# Autodesk Inventor assembly: Montagem Completa
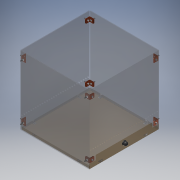
[picture p0: Inventor's stored thumbnail of the model, 180x180]
Saved by Autodesk Inventor 2018 (Build 220112000, 112)
## iProperties
Created: 2018-07-09
Part Number: Montagem Completa
Material: Genérico
Document SubType Name: Assembly
Designer: Regner
Author: Regner
## Documents named in this file (3)
- C:\Users\Regner\Documents\ROBOTA\2018\Tortura Ratos\Montagem Completa.iam
- C:\Users\Regner\Documents\ROBOTA\2018\Tortura Ratos\Gaveta.iam
- C:\Users\Regner\Documents\ROBOTA\2018\Tortura Ratos\Montagem Lateral.iam
## Components (2 placed, 2 different names)
1. Gaveta:1 [sub-assembly] — Coincidência:1, Alinhamento:1, Alinhamento:2, Alinhamento:3, Alinhamento:4, Alinhamento:5
2. Montagem Lateral:1 [sub-assembly] — Coincidência:1, Alinhamento:1, Alinhamento:2
## Relationships (6: Flush 5, Mate 1)
- Coincidência:1 [Mate]: Gaveta:1 ↔ Montagem Lateral:1
- Alinhamento:1 [Flush]: Gaveta:1 ↔ Montagem Lateral:1
- Alinhamento:2 [Flush]: Gaveta:1 ↔ Montagem Lateral:1
- Alinhamento:3 [Flush]: Gaveta:1
- Alinhamento:4 [Flush]: Gaveta:1
- Alinhamento:5 [Flush]: Gaveta:1
